# Autodesk Inventor assembly: CONTROLBOX2
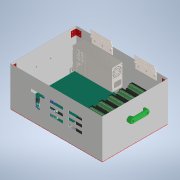
[picture p0: Inventor's stored thumbnail of the model, 180x180]
Saved by Autodesk Inventor 2020 (Build 240168000, 168)
## iProperties
Created: 2020-06-03
Part Number: CONTROLBOX2
Document SubType Name: Assembly
Designer: Gebruiker
Author: Gebruiker
## Documents named in this file (14)
- C:\Users\Gebruiker\Documents\GitHub\BeerMinder\3D-model\ControlBox\CONTROLBOX2.iam
- C:\Users\Gebruiker\Documents\GitHub\BeerMinder\3D-model\ControlBox\CONTROL_ONDERKANT.ipt
- C:\Users\Gebruiker\Documents\GitHub\BeerMinder\3D-model\ControlBox\CONTROL_LENGTE.ipt
- C:\Users\Gebruiker\Documents\GitHub\BeerMinder\3D-model\ControlBox\CONTROL_BREEDTE.ipt
- C:\Users\Gebruiker\Documents\GitHub\BeerMinder\3D-model\ControlBox\CONTOL_COMBI.ipt
- C:\Users\Gebruiker\Documents\GitHub\BeerMinder\3D-model\ControlBox\CONTROL_OPZETSTUK.ipt
- C:\Users\Gebruiker\Documents\GitHub\BeerMinder\3D-model\ControlBox\CONTROL_MONTEER.ipt
- C:\Users\Gebruiker\Documents\GitHub\BeerMinder\3D-model\ControlBox\controlbox_handvat.ipt
- C:\Users\Gebruiker\Documents\GitHub\BeerMinder\3D-model\ControlBox\ARDUINO DUE.iam
- C:\Users\Gebruiker\Documents\GitHub\BeerMinder\3D-model\ControlBox\Power supply unit.iam
- C:\Users\Gebruiker\Documents\GitHub\BeerMinder\3D-model\ControlBox\HY-DIV268N-5A.ipt
- C:\Users\Gebruiker\Documents\GitHub\BeerMinder\3D-model\ControlBox\DIN Rail 100 mm.ipt
- C:\Users\Gebruiker\Documents\GitHub\BeerMinder\3D-model\ControlBox\swithces\LM2596_Buck_Converter.ipt
- C:\Users\Gebruiker\Documents\GitHub\BeerMinder\3D-model\ControlBox\Biltema 25-539\Biltema 25-539.ipt
## Components (29 placed, 13 different names)
1. CONTROL_ONDERKANT:1 — Mate:1, Angle:1, Mate:2, Mate:3, Mate:6, Mate:37, Mate:38, Mate:41, Mate:44
2. CONTROL_LENGTE:1 — Mate:1, Angle:1, Mate:2, Mate:5, Mate:7, Mate:29, Mate:32, Mate:39, Mate:45, Angle:4, Angle:5, Angle:6, Angle:7, Angle:8, Angle:9
3. CONTROL_LENGTE:2 — Mate:3, Flush:1, Mate:25, Mate:28, Mate:36, Mate:42, Mate:59, Angle:10, Mate:64, Mate:65, Angle:15, Angle:16
4. CONTROL_BREEDTE:1 — Mate:5, Flush:1, Mate:27, Mate:30, Mate:34, Angle:3, Mate:43, Mate:46, Angle:12, Angle:13
5. CONTROL_BREEDTE:2 — Mate:6, Mate:7, Mate:26, Mate:31, Mate:33, Angle:2, Mate:35, Mate:40
6. CONTOL_COMBI:1 — Mate:44, Mate:45, Mate:46, Mate:47
7. CONTOL_COMBI:2 — Mate:41, Mate:42, Mate:43, Mate:50, Mate:51
8. CONTOL_COMBI:3 — Mate:38, Mate:39, Mate:40, Mate:48
9. CONTOL_COMBI:4 — Mate:35, Mate:36, Mate:37, Mate:49, Mate:52
10. CONTROL_OPZETSTUK:1 — Mate:47, Mate:48, Mate:49, Mate:50, Mate:51, Mate:52, Mate:53, Mate:54, Mate:55, Mate:56, Mate:57, Mate:58, Mate:60, Mate:61, Mate:62, Mate:63
11. CONTROL_MONTEER:1 — Mate:25, Mate:26
12. CONTROL_MONTEER:2 — Mate:27, Mate:28
13. CONTROL_MONTEER:3 — Mate:29, Mate:30
14. CONTROL_MONTEER:4 — Mate:31, Mate:32
15. controlbox_handvat:1 — Mate:34, Angle:3, Angle:11
16. controlbox_handvat:2 — Mate:33, Angle:2
17. ARDUINO DUE:1 [sub-assembly] — Mate:60, Angle:11, Angle:14
18. Power supply unit:1 [sub-assembly] — Mate:59, Angle:10
19. HY-DIV268N-5A:1 — Mate:53, Angle:4, Flush:2, Flush:6
20. HY-DIV268N-5A:2 — Mate:54, Angle:5, Flush:2, Flush:3, Flush:6
21. HY-DIV268N-5A:3 — Mate:55, Angle:6, Flush:3, Flush:4
22. HY-DIV268N-5A:4 — Mate:56, Angle:7, Flush:4, Flush:5
23. HY-DIV268N-5A:5 — Mate:57, Angle:8, Flush:5, Flush:7
24. HY-DIV268N-5A:6 — Mate:58, Angle:9, Flush:7
25. DIN Rail 100 mm:1 — Mate:62, Angle:13, Flush:8
26. DIN Rail 100 mm:2 — Mate:61, Angle:12, Flush:8
27. LM2596_Buck_Converter:1 — Mate:63, Angle:14
28. Biltema 25-539:1 — Mate:64, Angle:16, Flush:9
29. Biltema 25-539:2 — Mate:65, Angle:15, Flush:9
## Relationships (72: Mate 47, Angle 16, Flush 9)
- Mate:1: CONTROL_ONDERKANT:1 ↔ CONTROL_LENGTE:1
- Angle:1 (0 deg): CONTROL_ONDERKANT:1 ↔ CONTROL_LENGTE:1
- Mate:2: CONTROL_ONDERKANT:1 ↔ CONTROL_LENGTE:1
- Mate:3: CONTROL_ONDERKANT:1 ↔ CONTROL_LENGTE:2
- Mate:5: CONTROL_LENGTE:1 ↔ CONTROL_BREEDTE:1
- Flush:1: CONTROL_LENGTE:2 ↔ CONTROL_BREEDTE:1
- Mate:6: CONTROL_ONDERKANT:1 ↔ CONTROL_BREEDTE:2
- Mate:7: CONTROL_LENGTE:1 ↔ CONTROL_BREEDTE:2
- Mate:25: CONTROL_LENGTE:2 ↔ CONTROL_MONTEER:1
- Mate:26: CONTROL_BREEDTE:2 ↔ CONTROL_MONTEER:1
- Mate:27: CONTROL_BREEDTE:1 ↔ CONTROL_MONTEER:2
- Mate:28: CONTROL_LENGTE:2 ↔ CONTROL_MONTEER:2
- Mate:29: CONTROL_LENGTE:1 ↔ CONTROL_MONTEER:3
- Mate:30: CONTROL_BREEDTE:1 ↔ CONTROL_MONTEER:3
- Mate:31: CONTROL_BREEDTE:2 ↔ CONTROL_MONTEER:4
- Mate:32: CONTROL_LENGTE:1 ↔ CONTROL_MONTEER:4
- Mate:33: CONTROL_BREEDTE:2 ↔ controlbox_handvat:2
- Angle:2 (0 deg): CONTROL_BREEDTE:2 ↔ controlbox_handvat:2
- Mate:34: CONTROL_BREEDTE:1 ↔ controlbox_handvat:1
- Angle:3 (0 deg): CONTROL_BREEDTE:1 ↔ controlbox_handvat:1
- Mate:35: CONTROL_BREEDTE:2 ↔ CONTOL_COMBI:4
- Mate:36: CONTROL_LENGTE:2 ↔ CONTOL_COMBI:4
- Mate:37: CONTROL_ONDERKANT:1 ↔ CONTOL_COMBI:4
- Mate:38: CONTROL_ONDERKANT:1 ↔ CONTOL_COMBI:3
- Mate:39: CONTROL_LENGTE:1 ↔ CONTOL_COMBI:3
- Mate:40: CONTROL_BREEDTE:2 ↔ CONTOL_COMBI:3
- Mate:41: CONTROL_ONDERKANT:1 ↔ CONTOL_COMBI:2
- Mate:42: CONTROL_LENGTE:2 ↔ CONTOL_COMBI:2
- Mate:43: CONTROL_BREEDTE:1 ↔ CONTOL_COMBI:2
- Mate:44: CONTROL_ONDERKANT:1 ↔ CONTOL_COMBI:1
- Mate:45: CONTROL_LENGTE:1 ↔ CONTOL_COMBI:1
- Mate:46: CONTROL_BREEDTE:1 ↔ CONTOL_COMBI:1
- Mate:47: CONTOL_COMBI:1 ↔ CONTROL_OPZETSTUK:1
- Mate:48: CONTOL_COMBI:3 ↔ CONTROL_OPZETSTUK:1
- Mate:49: CONTOL_COMBI:4 ↔ CONTROL_OPZETSTUK:1
- Mate:50 (3 mm): CONTOL_COMBI:2 ↔ CONTROL_OPZETSTUK:1
- Mate:51 (3 mm): CONTOL_COMBI:2 ↔ CONTROL_OPZETSTUK:1
- Mate:52 (3 mm): CONTOL_COMBI:4 ↔ CONTROL_OPZETSTUK:1
- Mate:53: CONTROL_OPZETSTUK:1 ↔ HY-DIV268N-5A:1
- Angle:4 (0 deg): CONTROL_LENGTE:1 ↔ HY-DIV268N-5A:1
- Mate:54: CONTROL_OPZETSTUK:1 ↔ HY-DIV268N-5A:2
- Angle:5 (0 deg): CONTROL_LENGTE:1 ↔ HY-DIV268N-5A:2
- Mate:55: CONTROL_OPZETSTUK:1 ↔ HY-DIV268N-5A:3
- Angle:6 (0 deg): CONTROL_LENGTE:1 ↔ HY-DIV268N-5A:3
- Mate:56: CONTROL_OPZETSTUK:1 ↔ HY-DIV268N-5A:4
- Angle:7 (0 deg): CONTROL_LENGTE:1 ↔ HY-DIV268N-5A:4
- Mate:57: CONTROL_OPZETSTUK:1 ↔ HY-DIV268N-5A:5
- Angle:8 (0 deg): CONTROL_LENGTE:1 ↔ HY-DIV268N-5A:5
- Flush:2: HY-DIV268N-5A:1 ↔ HY-DIV268N-5A:2
- Flush:3: HY-DIV268N-5A:2 ↔ HY-DIV268N-5A:3
- Flush:4: HY-DIV268N-5A:3 ↔ HY-DIV268N-5A:4
- Flush:5: HY-DIV268N-5A:4 ↔ HY-DIV268N-5A:5
- Flush:6: HY-DIV268N-5A:1 ↔ HY-DIV268N-5A:2
- Mate:58: CONTROL_OPZETSTUK:1 ↔ HY-DIV268N-5A:6
- Angle:9 (0 deg): CONTROL_LENGTE:1 ↔ HY-DIV268N-5A:6
- Flush:7: HY-DIV268N-5A:5 ↔ HY-DIV268N-5A:6
- Mate:59: CONTROL_LENGTE:2 ↔ Power supply unit:1
- Angle:10 (0 deg): CONTROL_LENGTE:2 ↔ Power supply unit:1
- Mate:60: CONTROL_OPZETSTUK:1 ↔ ARDUINO DUE:1
- Angle:11 (0 deg): controlbox_handvat:1 ↔ ARDUINO DUE:1
- Mate:61: CONTROL_OPZETSTUK:1 ↔ DIN Rail 100 mm:2
- Mate:62: CONTROL_OPZETSTUK:1 ↔ DIN Rail 100 mm:1
- Angle:12 (0 deg): CONTROL_BREEDTE:1 ↔ DIN Rail 100 mm:2
- Angle:13 (0 deg): CONTROL_BREEDTE:1 ↔ DIN Rail 100 mm:1
- Flush:8: DIN Rail 100 mm:1 ↔ DIN Rail 100 mm:2
- Mate:63: CONTROL_OPZETSTUK:1 ↔ LM2596_Buck_Converter:1
- Angle:14 (0 deg): ARDUINO DUE:1 ↔ LM2596_Buck_Converter:1
- Mate:64: CONTROL_LENGTE:2 ↔ Biltema 25-539:1
- Mate:65: CONTROL_LENGTE:2 ↔ Biltema 25-539:2
- Angle:15 (0 deg): CONTROL_LENGTE:2 ↔ Biltema 25-539:2
- Angle:16 (0 deg): CONTROL_LENGTE:2 ↔ Biltema 25-539:1
- Flush:9: Biltema 25-539:1 ↔ Biltema 25-539:2
